# Autodesk Inventor assembly: Lego_Example
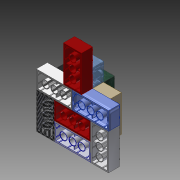
[picture p0: Inventor's stored thumbnail of the model, 180x180]
Saved by Autodesk Inventor 2015 (Build 190159000, 159)
## iProperties
Created: 2015-02-04
Part Number: Lego_Example
Document SubType Name: Assembly
Designer: Paul
Author: Paul
## Documents named in this file (2)
- C:\Users\Paul\Google Drive\All #ResBaz Shared\Paul2AlizaCAD\05_Assemby\03_Lego\Lego_Example.iam
- C:\Users\Paul\Google Drive\All #ResBaz Shared\Paul2AlizaCAD\05_Assemby\03_Lego\Lego_Brick.ipt
## Components (12 placed, 1 different names)
1. Lego_Brick:1 — Flush:1, Flush:2, Mate:1, Flush:3, Mate:3, Flush:7, Mate:7, Flush:10, Mate:8, Mate:9, Flush:11
2. Lego_Brick:2 — Flush:1, Flush:2, Mate:1, Mate:2, Mate:4, Flush:4, Flush:9, Mate:11, Flush:12
3. Lego_Brick:3 — Mate:4, Flush:4, Flush:5
4. Lego_Brick:4 — Mate:5, Flush:6, Flush:7, Mate:15, Flush:15
5. Lego_Brick:5 — Mate:6, Flush:8, Flush:9
6. Lego_Brick:6 — Flush:3, Mate:2, Mate:3, Flush:5, Mate:5, Flush:6, Mate:6, Flush:8, Flush:14, Mate:16, Flush:16, Mate:17
7. Lego_Brick:7 — Mate:7, Flush:10, Mate:8, Mate:10, Mate:12, Mate:14
8. Lego_Brick:8 — Mate:9, Mate:10, Flush:11, Mate:13
9. Lego_Brick:9 — Mate:11, Flush:12, Mate:12, Flush:13
10. Lego_Brick:10 — Mate:13, Flush:13, Mate:14
11. Lego_Brick:11 — Flush:14, Mate:15, Mate:16
12. Lego_Brick:12 — Flush:15, Flush:16, Mate:17
## Relationships (33: Mate 17, Flush 16)
- Flush:1: Lego_Brick:1 ↔ Lego_Brick:2
- Flush:2: Lego_Brick:1 ↔ Lego_Brick:2
- Mate:1: Lego_Brick:1 ↔ Lego_Brick:2
- Flush:3: Lego_Brick:1 ↔ Lego_Brick:6
- Mate:2: Lego_Brick:2 ↔ Lego_Brick:6
- Mate:3 (-7.874 mm): Lego_Brick:1 ↔ Lego_Brick:6
- Mate:4: Lego_Brick:2 ↔ Lego_Brick:3
- Flush:4: Lego_Brick:2 ↔ Lego_Brick:3
- Flush:5: Lego_Brick:3 ↔ Lego_Brick:6
- Mate:5: Lego_Brick:4 ↔ Lego_Brick:6
- Flush:6: Lego_Brick:4 ↔ Lego_Brick:6
- Flush:7: Lego_Brick:1 ↔ Lego_Brick:4
- Mate:6: Lego_Brick:5 ↔ Lego_Brick:6
- Flush:8: Lego_Brick:5 ↔ Lego_Brick:6
- Flush:9: Lego_Brick:2 ↔ Lego_Brick:5
- Mate:7: Lego_Brick:1 ↔ Lego_Brick:7
- Flush:10: Lego_Brick:1 ↔ Lego_Brick:7
- Mate:8 (-15.875 mm): Lego_Brick:1 ↔ Lego_Brick:7
- Mate:9: Lego_Brick:1 ↔ Lego_Brick:8
- Mate:10: Lego_Brick:7 ↔ Lego_Brick:8
- Flush:11: Lego_Brick:1 ↔ Lego_Brick:8
- Mate:11: Lego_Brick:2 ↔ Lego_Brick:9
- Flush:12: Lego_Brick:2 ↔ Lego_Brick:9
- Mate:12: Lego_Brick:7 ↔ Lego_Brick:9
- Mate:13: Lego_Brick:8 ↔ Lego_Brick:10
- Flush:13: Lego_Brick:9 ↔ Lego_Brick:10
- Mate:14: Lego_Brick:7 ↔ Lego_Brick:10
- Flush:14: Lego_Brick:6 ↔ Lego_Brick:11
- Mate:15: Lego_Brick:4 ↔ Lego_Brick:11
- Mate:16: Lego_Brick:6 ↔ Lego_Brick:11
- Flush:15: Lego_Brick:4 ↔ Lego_Brick:12
- Flush:16: Lego_Brick:6 ↔ Lego_Brick:12
- Mate:17: Lego_Brick:6 ↔ Lego_Brick:12
